# Autodesk Inventor assembly: Base
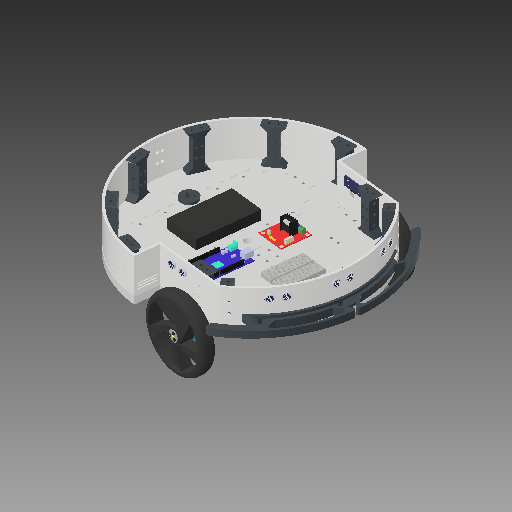
[picture p0: Inventor's stored thumbnail of the model, 512x512]
Saved by Autodesk Inventor 2017 SP1 (Build 210196100, 196)
## iProperties
Created: 2017-03-11
Part Number: Base
Document SubType Name: Assembly
Designer: zallen
Author: zallen
## Documents named in this file (10)
- C:\Users\Zach\Documents\GitHub\cr-laundry-robot\src\Base\Base.iam
- C:\Users\Zach\Documents\GitHub\cr-laundry-robot\src\Base\Swivel Wheel.ipt
- C:\Users\Zach\Documents\GitHub\cr-laundry-robot\lib\Breadboard\breadboard_350_pos_asm.iam
- C:\Users\Zach\Documents\GitHub\cr-laundry-robot\lib\Arduino Mega 2560\Arduino Mega 2560.ipt
- C:\Users\Zach\Documents\GitHub\cr-laundry-robot\lib\L298n\Драйвер двигателей L298N.ipt
- C:\Users\Zach\Documents\GitHub\cr-laundry-robot\src\Base\Drive Wheel Assembly\DriveAssembly.iam
- C:\Users\Zach\Documents\GitHub\cr-laundry-robot\src\Base\Battery Pack Assembly\BatteryPackAssembly.iam
- C:\Users\Zach\Documents\GitHub\cr-laundry-robot\src\Base\Bumper Assembly\Bumper Assembly.iam
- C:\Users\Zach\Documents\GitHub\cr-laundry-robot\src\Base\Chassis - Modular\Chassis.iam
- C:\Users\Zach\Documents\GitHub\cr-laundry-robot\lib\HC-SR04 Ultasonic Sensor\Sensor Ultrasónico.ipt
## Components (13 placed, 9 different names)
1. Swivel Wheel:1 — Mate:75, Mate:76
2. breadboard_350_pos_asm:1 [sub-assembly] — Mate:89, Mate:92, Mate:94
3. Arduino Mega 2560:1 — Mate:90, Mate:91, Mate:98
4. L298N:1 — Mate:95, Mate:96, Mate:97
5. DriveAssembly:1 [sub-assembly] — Mate:72, Mate:74, Mate:103
6. BatteryPackAssembly:1 [sub-assembly] — Mate:99, Mate:100, Mate:106
7. Bumper Assembly:1 [sub-assembly] — Mate:67, Mate:104, Mate:105
8. Chassis:1 [sub-assembly] — Mate:66, Mate:67, Mate:72, Mate:74, Mate:75, Mate:76, Mate:89, Mate:90, Mate:91, Mate:92, Mate:94, Mate:95, Mate:96, Mate:97, Mate:98, Mate:99, Mate:100, Mate:103, Mate:104, Mate:105, Mate:106, Mate:107, Mate:108, Mate:109, Mate:110, Mate:111, Mate:112, Mate:113, Mate:114, Mate:115, Mate:116, Mate:117, Mate:118, Tangent:1, Tangent:2, Tangent:3
9. Sensor Ultrasónico:1 — Mate:107, Mate:108, Mate:109
10. Sensor Ultrasónico:2 — Mate:110, Mate:111, Mate:112
11. Sensor Ultrasónico:3 — Mate:113, Mate:114, Tangent:3
12. Sensor Ultrasónico:4 — Mate:115, Mate:116, Tangent:2
13. Sensor Ultrasónico:5 — Mate:117, Mate:118, Tangent:1
## Relationships (36: Mate 33, Tangent 3)
- Mate:66: Chassis:1
- Mate:67: Bumper Assembly:1 ↔ Chassis:1
- Mate:72: DriveAssembly:1 ↔ Chassis:1
- Mate:74: DriveAssembly:1 ↔ Chassis:1
- Mate:75: Swivel Wheel:1 ↔ Chassis:1
- Mate:76: Swivel Wheel:1 ↔ Chassis:1
- Mate:89: breadboard_350_pos_asm:1 ↔ Chassis:1
- Mate:90: Arduino Mega 2560:1 ↔ Chassis:1
- Mate:91: Arduino Mega 2560:1 ↔ Chassis:1
- Mate:92: breadboard_350_pos_asm:1 ↔ Chassis:1
- Mate:94: breadboard_350_pos_asm:1 ↔ Chassis:1
- Mate:95: L298N:1 ↔ Chassis:1
- Mate:96: L298N:1 ↔ Chassis:1
- Mate:97: L298N:1 ↔ Chassis:1
- Mate:98: Arduino Mega 2560:1 ↔ Chassis:1
- Mate:99: BatteryPackAssembly:1 ↔ Chassis:1
- Mate:100: BatteryPackAssembly:1 ↔ Chassis:1
- Mate:103: DriveAssembly:1 ↔ Chassis:1
- Mate:104: Bumper Assembly:1 ↔ Chassis:1
- Mate:105: Bumper Assembly:1 ↔ Chassis:1
- Mate:106: BatteryPackAssembly:1 ↔ Chassis:1
- Mate:107: Chassis:1 ↔ Sensor Ultrasónico:1
- Mate:108: Chassis:1 ↔ Sensor Ultrasónico:1
- Mate:109: Chassis:1 ↔ Sensor Ultrasónico:1
- Mate:110: Chassis:1 ↔ Sensor Ultrasónico:2
- Mate:111: Chassis:1 ↔ Sensor Ultrasónico:2
- Mate:112: Chassis:1 ↔ Sensor Ultrasónico:2
- Mate:113: Chassis:1 ↔ Sensor Ultrasónico:3
- Mate:114: Chassis:1 ↔ Sensor Ultrasónico:3
- Mate:115: Chassis:1 ↔ Sensor Ultrasónico:4
- Mate:116: Chassis:1 ↔ Sensor Ultrasónico:4
- Mate:117: Chassis:1 ↔ Sensor Ultrasónico:5
- Mate:118: Chassis:1 ↔ Sensor Ultrasónico:5
- Tangent:1: Chassis:1 ↔ Sensor Ultrasónico:5
- Tangent:2: Chassis:1 ↔ Sensor Ultrasónico:4
- Tangent:3: Chassis:1 ↔ Sensor Ultrasónico:3
